# Autodesk Inventor assembly: KosselCNC1515_Vertex_Lower
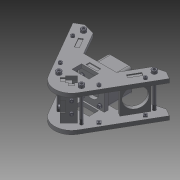
[picture p0: Inventor's stored thumbnail of the model, 180x180]
Saved by Autodesk Inventor 2014 (Build 180170000, 170)
## iProperties
Created: 2014-08-25
Part Number: KosselCNC1515_Vertex_Lower
Document SubType Name: Assembly
Designer: ThatOtherGuy
Author: ThatOtherGuy
## Documents named in this file (14)
- U:\Hobbies\Inventor\KosselCNC1515\Frame\KosselCNC1515_Vertex_Lower.iam
- U:\Hobbies\Inventor\KosselCNC1515\Frame\Frame_Lower_Plate_Bottom.ipt
- U:\Hobbies\Inventor\KosselCNC1515\Frame\Frame_Lower_Plate_Motor.ipt
- U:\Hobbies\Inventor\KosselCNC1515\NEMA17.ipt
- U:\Hobbies\Inventor\KosselCNC1515\Frame\Frame_Lower_Vertical_Plate_A.ipt
- U:\Hobbies\Inventor\KosselCNC1515\Frame\Frame_Lower_Vertical_Plate_B.ipt
- U:\Hobbies\Inventor\KosselCNC1515\Frame\Frame_Lower_Vertical_Plate_C.ipt
- U:\Hobbies\Inventor\Content Center Files\R2014\en-US\ANSI B18.3.1M(1)\ANSI B18.3.1M - M5x0.8 x 70(2).ipt
- U:\Hobbies\Inventor\Content Center Files\R2014\en-US\ANSI B18.3.1M(1)\ANSI B18.3.1M - M3x0.5 x 10(2).ipt
- U:\Hobbies\Inventor\Content Center Files\R2014\en-US\ISO 10511\ISO 10511 - M5.ipt
- U:\Hobbies\Inventor\Content Center Files\R2014\en-US\DIN 562\DIN 562 - M3 x 5.5.ipt
- U:\Hobbies\Inventor\Content Center Files\R2014\en-US\DIN 125-1  A\DIN 125 - A 3.2.ipt
- U:\Hobbies\Inventor\Content Center Files\R2014\en-US\ANSI B18.3.1M(1)\ANSI B18.3.1M - M3x0.5 x 12(2).ipt
- U:\Hobbies\Inventor\Content Center Files\R2014\en-US\DIN 125-1  A\DIN 125 - A 5.3.ipt
## Components (52 placed, 13 different names)
1. Frame_Lower_Plate_Bottom:1 — Mate:10, Mate:11, Mate:12, Mate:13, Mate:14, Mate:15, Mate:16, Mate:17, Mate:18, Mate:19, Mate:20, Mate:21, Mate:22, Mate:23, Mate:24, Insert:5, Insert:6, Insert:7, Insert:8, Insert:17, Insert:18, Insert:19, Insert:20, Insert:41, Insert:42, Insert:43, Insert:44
2. Frame_Lower_Vertical_Plate_A:1 — Mate:10, Mate:11, Mate:12, Insert:9, Insert:10, Insert:29, Insert:30
3. Frame_Lower_Vertical_Plate_B:1 — Mate:13, Mate:14, Mate:15, Insert:11, Insert:12, Insert:31, Insert:32
4. Frame_Lower_Vertical_Plate_C:1 — Mate:16, Mate:17, Mate:18
5. Frame_Lower_Vertical_Plate_C:2 — Mate:19, Mate:20, Mate:21
6. Frame_Lower_Plate_Motor:1 — Mate:22, Mate:23, Mate:24, Mate:25, Mate:26, Mate:27, Mate:28, Mate:29, Mate:30, Insert:25, Insert:26, Insert:27, Insert:28, Mate:47, Mate:49, Mate:51, Mate:53
7. NEMA17:1 — Mate:25, Mate:26, Mate:27
8. Frame_Lower_Plate_Bottom:2 — Mate:28, Mate:29, Mate:30, Insert:13, Insert:16, Insert:21, Insert:22, Insert:33, Insert:34, Insert:35, Insert:36, Insert:37, Insert:38, Insert:39, Insert:40
9. DIN 125-1 A A 5.3:1 — Insert:41, Insert:45
10. DIN 125-1 A A 5.3:2 — Insert:42, Insert:46
11. DIN 125-1 A A 5.3:3 — Insert:43, Insert:47
12. DIN 125-1 A A 5.3:4 — Insert:44, Insert:48
13. DIN EN ISO 10511 M5:1 — Insert:45
14. DIN EN ISO 10511 M5:2 — Insert:46
15. DIN EN ISO 10511 M5:3 — Insert:47
16. DIN EN ISO 10511 M5:4 — Insert:48
17. DIN 562 M3:13 — Insert:33
18. DIN 562 M3:14 — Insert:34
19. Broached Socket Head Cap Screw - Metric M3x0.5 x 10:13 — Insert:35
20. Broached Socket Head Cap Screw - Metric M3x0.5 x 10:14 — Insert:36
21. Broached Socket Head Cap Screw - Metric M5x0.8 x 70:1 — Insert:37
22. Broached Socket Head Cap Screw - Metric M5x0.8 x 70:2 — Insert:38
23. Broached Socket Head Cap Screw - Metric M5x0.8 x 70:3 — Insert:39
24. Broached Socket Head Cap Screw - Metric M5x0.8 x 70:4 — Insert:40
25. DIN 562 M3:9 — Insert:29
26. DIN 562 M3:10 — Insert:30
27. DIN 562 M3:11 — Insert:31
28. DIN 562 M3:12 — Insert:32
29. Broached Socket Head Cap Screw - Metric M3x0.5 x 10:1 — Insert:5
30. Broached Socket Head Cap Screw - Metric M3x0.5 x 10:2 — Insert:6
31. Broached Socket Head Cap Screw - Metric M3x0.5 x 10:3 — Insert:7
32. Broached Socket Head Cap Screw - Metric M3x0.5 x 10:4 — Insert:8
33. Broached Socket Head Cap Screw - Metric M3x0.5 x 10:5 — Insert:9
34. Broached Socket Head Cap Screw - Metric M3x0.5 x 10:6 — Insert:10
35. Broached Socket Head Cap Screw - Metric M3x0.5 x 10:7 — Insert:11
36. Broached Socket Head Cap Screw - Metric M3x0.5 x 10:8 — Insert:12
37. Broached Socket Head Cap Screw - Metric M3x0.5 x 10:9 — Insert:13
38. Broached Socket Head Cap Screw - Metric M3x0.5 x 10:12 — Insert:16
39. DIN 562 M3:1 — Insert:17
40. DIN 562 M3:2 — Insert:18
41. DIN 562 M3:3 — Insert:19
42. DIN 562 M3:4 — Insert:20
43. DIN 562 M3:5 — Insert:21
44. DIN 562 M3:6 — Insert:22
45. DIN 125-1 A A 3.2:1 — Insert:25, Mate:48, Mate:50, Mate:52, Mate:54
46. DIN 125-1 A A 3.2:2 — Insert:26
47. DIN 125-1 A A 3.2:3 — Insert:27
48. DIN 125-1 A A 3.2:4 — Insert:28
49. Broached Socket Head Cap Screw - Metric M3x0.5 x 12:1 — Mate:47, Mate:48
50. Broached Socket Head Cap Screw - Metric M3x0.5 x 12:2 — Mate:49, Mate:50
51. Broached Socket Head Cap Screw - Metric M3x0.5 x 12:3 — Mate:51, Mate:52
52. Broached Socket Head Cap Screw - Metric M3x0.5 x 12:4 — Mate:53, Mate:54
## Relationships (69: Insert 40, Mate 29)
- Mate:10: Frame_Lower_Plate_Bottom:1 ↔ Frame_Lower_Vertical_Plate_A:1
- Mate:11: Frame_Lower_Plate_Bottom:1 ↔ Frame_Lower_Vertical_Plate_A:1
- Mate:12: Frame_Lower_Plate_Bottom:1 ↔ Frame_Lower_Vertical_Plate_A:1
- Mate:13: Frame_Lower_Plate_Bottom:1 ↔ Frame_Lower_Vertical_Plate_B:1
- Mate:14: Frame_Lower_Plate_Bottom:1 ↔ Frame_Lower_Vertical_Plate_B:1
- Mate:15: Frame_Lower_Plate_Bottom:1 ↔ Frame_Lower_Vertical_Plate_B:1
- Mate:16: Frame_Lower_Plate_Bottom:1 ↔ Frame_Lower_Vertical_Plate_C:1
- Mate:17: Frame_Lower_Plate_Bottom:1 ↔ Frame_Lower_Vertical_Plate_C:1
- Mate:18: Frame_Lower_Plate_Bottom:1 ↔ Frame_Lower_Vertical_Plate_C:1
- Mate:19: Frame_Lower_Plate_Bottom:1 ↔ Frame_Lower_Vertical_Plate_C:2
- Mate:20: Frame_Lower_Plate_Bottom:1 ↔ Frame_Lower_Vertical_Plate_C:2
- Mate:21: Frame_Lower_Plate_Bottom:1 ↔ Frame_Lower_Vertical_Plate_C:2
- Mate:22: Frame_Lower_Plate_Bottom:1 ↔ Frame_Lower_Plate_Motor:1
- Mate:23: Frame_Lower_Plate_Bottom:1 ↔ Frame_Lower_Plate_Motor:1
- Mate:24: Frame_Lower_Plate_Bottom:1 ↔ Frame_Lower_Plate_Motor:1
- Mate:25: Frame_Lower_Plate_Motor:1 ↔ NEMA17:1
- Mate:26: Frame_Lower_Plate_Motor:1 ↔ NEMA17:1
- Mate:27: Frame_Lower_Plate_Motor:1 ↔ NEMA17:1
- Mate:28: Frame_Lower_Plate_Motor:1 ↔ Frame_Lower_Plate_Bottom:2
- Mate:29: Frame_Lower_Plate_Motor:1 ↔ Frame_Lower_Plate_Bottom:2
- Mate:30: Frame_Lower_Plate_Motor:1 ↔ Frame_Lower_Plate_Bottom:2
- Insert:5: Frame_Lower_Plate_Bottom:1 ↔ Broached Socket Head Cap Screw - Metric M3x0.5 x 10:1
- Insert:6: Frame_Lower_Plate_Bottom:1 ↔ Broached Socket Head Cap Screw - Metric M3x0.5 x 10:2
- Insert:7: Frame_Lower_Plate_Bottom:1 ↔ Broached Socket Head Cap Screw - Metric M3x0.5 x 10:3
- Insert:8: Frame_Lower_Plate_Bottom:1 ↔ Broached Socket Head Cap Screw - Metric M3x0.5 x 10:4
- Insert:9: Frame_Lower_Vertical_Plate_A:1 ↔ Broached Socket Head Cap Screw - Metric M3x0.5 x 10:5
- Insert:10: Frame_Lower_Vertical_Plate_A:1 ↔ Broached Socket Head Cap Screw - Metric M3x0.5 x 10:6
- Insert:11: Frame_Lower_Vertical_Plate_B:1 ↔ Broached Socket Head Cap Screw - Metric M3x0.5 x 10:7
- Insert:12: Frame_Lower_Vertical_Plate_B:1 ↔ Broached Socket Head Cap Screw - Metric M3x0.5 x 10:8
- Insert:13: Frame_Lower_Plate_Bottom:2 ↔ Broached Socket Head Cap Screw - Metric M3x0.5 x 10:9
- Insert:16: Frame_Lower_Plate_Bottom:2 ↔ Broached Socket Head Cap Screw - Metric M3x0.5 x 10:12
- Insert:17: Frame_Lower_Plate_Bottom:1 ↔ DIN 562 M3:1
- Insert:18: Frame_Lower_Plate_Bottom:1 ↔ DIN 562 M3:2
- Insert:19: Frame_Lower_Plate_Bottom:1 ↔ DIN 562 M3:3
- Insert:20: Frame_Lower_Plate_Bottom:1 ↔ DIN 562 M3:4
- Insert:21: Frame_Lower_Plate_Bottom:2 ↔ DIN 562 M3:5
- Insert:22: Frame_Lower_Plate_Bottom:2 ↔ DIN 562 M3:6
- Insert:25: Frame_Lower_Plate_Motor:1 ↔ DIN 125-1 A A 3.2:1
- Insert:26: Frame_Lower_Plate_Motor:1 ↔ DIN 125-1 A A 3.2:2
- Insert:27: Frame_Lower_Plate_Motor:1 ↔ DIN 125-1 A A 3.2:3
- Insert:28: Frame_Lower_Plate_Motor:1 ↔ DIN 125-1 A A 3.2:4
- Mate:47: Frame_Lower_Plate_Motor:1 ↔ Broached Socket Head Cap Screw - Metric M3x0.5 x 12:1
- Mate:48: DIN 125-1 A A 3.2:1 ↔ Broached Socket Head Cap Screw - Metric M3x0.5 x 12:1
- Mate:49: Frame_Lower_Plate_Motor:1 ↔ Broached Socket Head Cap Screw - Metric M3x0.5 x 12:2
- Mate:50: DIN 125-1 A A 3.2:1 ↔ Broached Socket Head Cap Screw - Metric M3x0.5 x 12:2
- Mate:51: Frame_Lower_Plate_Motor:1 ↔ Broached Socket Head Cap Screw - Metric M3x0.5 x 12:3
- Mate:52: DIN 125-1 A A 3.2:1 ↔ Broached Socket Head Cap Screw - Metric M3x0.5 x 12:3
- Mate:53: Frame_Lower_Plate_Motor:1 ↔ Broached Socket Head Cap Screw - Metric M3x0.5 x 12:4
- Mate:54: DIN 125-1 A A 3.2:1 ↔ Broached Socket Head Cap Screw - Metric M3x0.5 x 12:4
- Insert:29: Frame_Lower_Vertical_Plate_A:1 ↔ DIN 562 M3:9
- Insert:30: Frame_Lower_Vertical_Plate_A:1 ↔ DIN 562 M3:10
- Insert:31: Frame_Lower_Vertical_Plate_B:1 ↔ DIN 562 M3:11
- Insert:32: Frame_Lower_Vertical_Plate_B:1 ↔ DIN 562 M3:12
- Insert:33: Frame_Lower_Plate_Bottom:2 ↔ DIN 562 M3:13
- Insert:34: Frame_Lower_Plate_Bottom:2 ↔ DIN 562 M3:14
- Insert:35: Frame_Lower_Plate_Bottom:2 ↔ Broached Socket Head Cap Screw - Metric M3x0.5 x 10:13
- Insert:36: Frame_Lower_Plate_Bottom:2 ↔ Broached Socket Head Cap Screw - Metric M3x0.5 x 10:14
- Insert:37: Frame_Lower_Plate_Bottom:2 ↔ Broached Socket Head Cap Screw - Metric M5x0.8 x 70:1
- Insert:38: Frame_Lower_Plate_Bottom:2 ↔ Broached Socket Head Cap Screw - Metric M5x0.8 x 70:2
- Insert:39: Frame_Lower_Plate_Bottom:2 ↔ Broached Socket Head Cap Screw - Metric M5x0.8 x 70:3
- Insert:40: Frame_Lower_Plate_Bottom:2 ↔ Broached Socket Head Cap Screw - Metric M5x0.8 x 70:4
- Insert:41: Frame_Lower_Plate_Bottom:1 ↔ DIN 125-1 A A 5.3:1
- Insert:42: Frame_Lower_Plate_Bottom:1 ↔ DIN 125-1 A A 5.3:2
- Insert:43: Frame_Lower_Plate_Bottom:1 ↔ DIN 125-1 A A 5.3:3
- Insert:44: Frame_Lower_Plate_Bottom:1 ↔ DIN 125-1 A A 5.3:4
- Insert:45: DIN 125-1 A A 5.3:1 ↔ DIN EN ISO 10511 M5:1
- Insert:46: DIN 125-1 A A 5.3:2 ↔ DIN EN ISO 10511 M5:2
- Insert:47: DIN 125-1 A A 5.3:3 ↔ DIN EN ISO 10511 M5:3
- Insert:48: DIN 125-1 A A 5.3:4 ↔ DIN EN ISO 10511 M5:4
